# Autodesk Inventor assembly: test-model-1
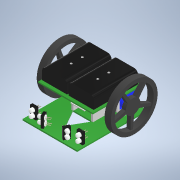
[picture p0: Inventor's stored thumbnail of the model, 180x180]
Saved by Autodesk Inventor 2022 (Build 260153000, 153)
## iProperties
Created: 2024-05-30
Part Number: test-model-1
Document SubType Name: Assembly
Designer: yamashita1
Author: yamashita1
## Documents named in this file (10)
- G:\マイドライブ\project\micro-mouse\3D-Model\test-model-1.iam
- G:\マイドライブ\project\micro-mouse\3D-Model\PCB-Bottom.ipt
- G:\マイドライブ\project\micro-mouse\3D-Model\FS90R.ipt
- G:\マイドライブ\project\micro-mouse\3D-Model\FS90R-W.ipt
- G:\マイドライブ\project\micro-mouse\3D-Model\PCB-main.ipt
- G:\マイドライブ\project\micro-mouse\3D-Model\FS90-Mount2.ipt
- G:\マイドライブ\project\micro-mouse\3D-Model\FS90-Mount2-Mirror.ipt
- G:\マイドライブ\project\micro-mouse\3D-Model\BH321-1P24.ipt
- G:\マイドライブ\project\micro-mouse\3D-Model\Photo-Sensor.iam
- G:\マイドライブ\project\micro-mouse\3D-Model\ESP32-DevKitC.ipt
## Components (15 placed, 9 different names)
1. PCB-Bottom:1 — フラッシュ:1, フラッシュ:2, フラッシュ:3, フラッシュ:4, メイト:8, メイト:10, フラッシュ:6, フラッシュ:7, メイト:13, メイト:14, メイト:16, メイト:25, メイト:26
2. FS90R:1 — フラッシュ:1, フラッシュ:2, 回転:1, メイト:8, フラッシュ:8, メイト:15
3. FS90R:2 — フラッシュ:3, フラッシュ:4, 回転:2, メイト:10, フラッシュ:9, メイト:17
4. FS90R-W:1 — 回転:1
5. FS90R-W:2 — 回転:2
6. PCB-main:1 — フラッシュ:6, フラッシュ:7, メイト:13, メイト:27, メイト:28, メイト:29, メイト:30, メイト:31
7. FS90-Mount2:1 — フラッシュ:8, メイト:14, メイト:15
8. FS90-Mount2-Mirror:1 — フラッシュ:9, メイト:16, メイト:17
9. BH321-1P24:1 — メイト:26
10. BH321-1P24:2 — メイト:25
11. Photo-Sensor:1 [sub-assembly] — メイト:27
12. Photo-Sensor:2 [sub-assembly] — メイト:28
13. Photo-Sensor:3 [sub-assembly] — メイト:29
14. Photo-Sensor:4 [sub-assembly] — メイト:30
15. ESP32-DevKitC:1 — メイト:31
## Relationships (24: Mate 14, Flush 8, RevoluteJoint 2)
- フラッシュ:1 [Flush]: PCB-Bottom:1 ↔ FS90R:1
- フラッシュ:2 [Flush] (8 mm): PCB-Bottom:1 ↔ FS90R:1
- フラッシュ:3 [Flush]: PCB-Bottom:1 ↔ FS90R:2
- フラッシュ:4 [Flush] (-8 mm): PCB-Bottom:1 ↔ FS90R:2
- 回転:1 [RevoluteJoint]: FS90R:1 ↔ FS90R-W:1
- 回転:2 [RevoluteJoint]: FS90R:2 ↔ FS90R-W:2
- メイト:8 [Mate]: PCB-Bottom:1 ↔ FS90R:1
- メイト:10 [Mate]: PCB-Bottom:1 ↔ FS90R:2
- フラッシュ:6 [Flush]: PCB-Bottom:1 ↔ PCB-main:1
- フラッシュ:7 [Flush]: PCB-Bottom:1 ↔ PCB-main:1
- メイト:13 [Mate] (30 mm): PCB-Bottom:1 ↔ PCB-main:1
- フラッシュ:8 [Flush]: FS90R:1 ↔ FS90-Mount2:1
- メイト:14 [Mate]: PCB-Bottom:1 ↔ FS90-Mount2:1
- メイト:15 [Mate] (0.2 mm): FS90R:1 ↔ FS90-Mount2:1
- フラッシュ:9 [Flush]: FS90R:2 ↔ FS90-Mount2-Mirror:1
- メイト:16 [Mate]: PCB-Bottom:1 ↔ FS90-Mount2-Mirror:1
- メイト:17 [Mate] (0.2 mm): FS90R:2 ↔ FS90-Mount2-Mirror:1
- メイト:25 [Mate]: PCB-Bottom:1 ↔ BH321-1P24:2
- メイト:26 [Mate]: PCB-Bottom:1 ↔ BH321-1P24:1
- メイト:27 [Mate]: PCB-main:1 ↔ Photo-Sensor:1
- メイト:28 [Mate]: PCB-main:1 ↔ Photo-Sensor:2
- メイト:29 [Mate]: PCB-main:1 ↔ Photo-Sensor:3
- メイト:30 [Mate]: PCB-main:1 ↔ Photo-Sensor:4
- メイト:31 [Mate]: PCB-main:1 ↔ ESP32-DevKitC:1
